# Autodesk Inventor assembly: ControlPanel
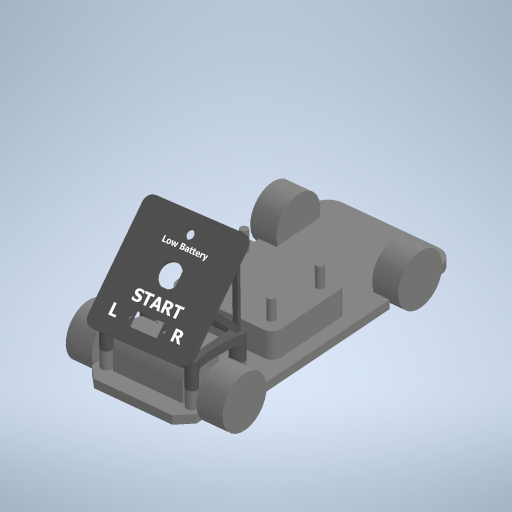
[picture p0: Inventor's stored thumbnail of the model, 512x512]
Saved by Autodesk Inventor 2024.2 (Build 282272000, 272)
## iProperties
Created: 2024-05-04
Part Number: ControlPanel
Document SubType Name: Assembly
Designer: ringl
Author: ringl
## Documents named in this file (6)
- C:\Users\ringl\OneDrive\Uni_PC_backup\Y4S2\EE579\Assignment\EE579-Skittles\CAD\Assembly\ControlPanel.iam
- C:\Users\ringl\OneDrive\Uni_PC_backup\Y4S2\EE579\Assignment\EE579-Skittles\CAD\Components\CarApproximation02.ipt
- C:\Users\ringl\OneDrive\Uni_PC_backup\Y4S2\EE579\Assignment\EE579-Skittles\CAD\ControlPanel_Bottom.ipt
- C:\Users\ringl\OneDrive\Uni_PC_backup\Y4S2\EE579\Assignment\EE579-Skittles\CAD\ControlPanel_Middle.ipt
- C:\Users\ringl\OneDrive\Uni_PC_backup\Y4S2\EE579\Assignment\EE579-Skittles\CAD\ControlPanel_Top.ipt
- C:\Users\ringl\OneDrive\Uni_PC_backup\Y4S2\EE579\Assignment\EE579-Skittles\CAD\Components\M2x16.ipt
## Components (7 placed, 5 different names)
1. CarApproximation02:1 — Mate:7, Mate:8, Mate:9, Mate:12, Mate:13, Mate:14, Mate:15
2. ControlPanel_Bottom:1 — Mate:1, Mate:2, Mate:3, Mate:4, Mate:5, Mate:6, Mate:7, Mate:8, Mate:9
3. ControlPanel_Middle:1 — Mate:1, Mate:2, Mate:5, Mate:10, Mate:11
4. ControlPanel_Middle:2 — Mate:3, Mate:4, Mate:6, Tangent:1
5. ControlPanel_Top:1 — Mate:10, Mate:11, Tangent:1
6. M2x16:1 — Mate:12, Mate:14
7. M2x16:2 — Mate:13, Mate:15
## Relationships (16: Mate 15, Tangent 1)
- Mate:1: ControlPanel_Bottom:1 ↔ ControlPanel_Middle:1
- Mate:2: ControlPanel_Bottom:1 ↔ ControlPanel_Middle:1
- Mate:3: ControlPanel_Bottom:1 ↔ ControlPanel_Middle:2
- Mate:4: ControlPanel_Bottom:1 ↔ ControlPanel_Middle:2
- Mate:5: ControlPanel_Bottom:1 ↔ ControlPanel_Middle:1
- Mate:6: ControlPanel_Bottom:1 ↔ ControlPanel_Middle:2
- Mate:7: CarApproximation02:1 ↔ ControlPanel_Bottom:1
- Mate:8: CarApproximation02:1 ↔ ControlPanel_Bottom:1
- Mate:9: CarApproximation02:1 ↔ ControlPanel_Bottom:1
- Mate:10: ControlPanel_Middle:1 ↔ ControlPanel_Top:1
- Mate:11 (3 mm): ControlPanel_Middle:1 ↔ ControlPanel_Top:1
- Tangent:1 (7 mm): ControlPanel_Middle:2 ↔ ControlPanel_Top:1
- Mate:12: CarApproximation02:1 ↔ M2x16:1
- Mate:13: CarApproximation02:1 ↔ M2x16:2
- Mate:14: CarApproximation02:1 ↔ M2x16:1
- Mate:15: CarApproximation02:1 ↔ M2x16:2
